# Autodesk Inventor assembly: Head_camera_cover
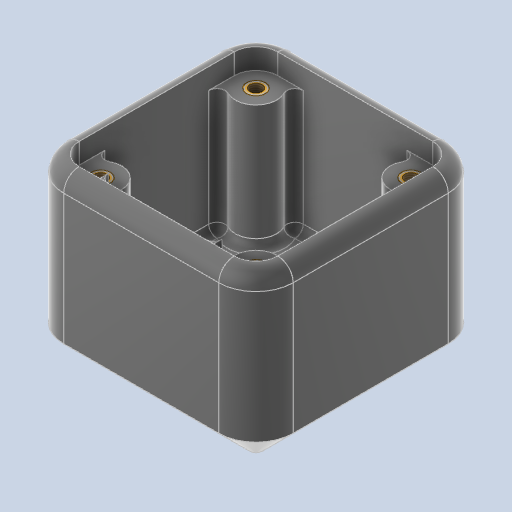
[picture p0: Inventor's stored thumbnail of the model, 512x512]
Saved by Autodesk Inventor 2022.3 (Build 263350000, 350)
## iProperties
Created: 2023-04-07
Part Number: Head_camera_cover
Document SubType Name: Assembly
Designer: Masato Kubotera
Author: Masato Kubotera
## Documents named in this file (3)
- C:\Users\Masato\Documents\Inventor\Inventor for CIT Brains\SUSTAINA-OP\UpperBody\Head\Head_camera_cover.iam
- C:\Users\Masato\Documents\Inventor\Inventor for CIT Brains\SUSTAINA-OP\UpperBody\Head\Head_camera_cover.ipt
- C:\Users\Masato\Documents\Inventor\Inventor for CIT Brains\SUSTAINA-OP\ReadyMade\InsertNut\UD-43040.ipt
## Components (5 placed, 2 different names)
1. Head_camera_cover:1 — 挿入:1, 挿入:2, 挿入:3, 挿入:4
2. UD-43040:1 — 挿入:1
3. UD-43040:2 — 挿入:2
4. UD-43040:3 — 挿入:3
5. UD-43040:4 — 挿入:4
## Relationships (4: Insert 4)
- 挿入:1 [Insert]: Head_camera_cover:1 ↔ UD-43040:1
- 挿入:2 [Insert]: Head_camera_cover:1 ↔ UD-43040:2
- 挿入:3 [Insert]: Head_camera_cover:1 ↔ UD-43040:3
- 挿入:4 [Insert]: Head_camera_cover:1 ↔ UD-43040:4
